# Autodesk Inventor assembly: Hand
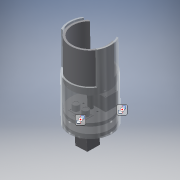
[picture p0: Inventor's stored thumbnail of the model, 180x180]
Saved by Autodesk Inventor 2016 (Build 200138000, 138)
## iProperties
Created: 2016-11-13
Part Number: Hand
Material: 一般
Document SubType Name: Assembly
Designer: Daisuke
Author: Daisuke
## Documents named in this file (10)
- C:\Users\Daisuke\Documents\GitHub\CAD\Hand\ver2\Hand.iam
- C:\Users\Daisuke\Documents\GitHub\CAD\Hand\ver2\Servo.iam
- C:\Users\Daisuke\Documents\GitHub\CAD\Hand\ver2\outsideBottom2.ipt
- C:\Users\Daisuke\Documents\GitHub\CAD\Hand\ver2\outsideBottom1.ipt
- C:\Users\Daisuke\Documents\GitHub\CAD\Hand\ver2\Servo.ipt
- C:\Users\Daisuke\Documents\GitHub\CAD\Hand\ver2\ServoArm.ipt
- C:\Users\Daisuke\Documents\GitHub\CAD\Hand\ver2\UFL08 -Housing.ipt
- C:\Users\Daisuke\Documents\GitHub\CAD\Hand\ver2\UltrasonicDistanceSencor.ipt
- C:\Users\Daisuke\Documents\GitHub\CAD\Hand\ver2\insideHand.iam
- C:\Users\Daisuke\Documents\GitHub\CAD\Hand\ver2\outsideCover1.ipt
## Components (9 placed, 8 different names)
1. Servo:1 [sub-assembly] — 挿入:1, 挿入:2, 挿入:3
2. outsideBottom2:1 — 挿入:9, 挿入:10, 挿入:11, メイト:1, メイト:4
3. outsideBottom1:1 — 挿入:1, 挿入:2, 挿入:3, 挿入:4, 挿入:5, 挿入:12, 挿入:13, メイト:2, メイト:3
4. Servo:2 — 挿入:8
5. ServoArm:1 — 挿入:8, 挿入:9, 挿入:10, 挿入:11
6. UFL08 -Housing:1 — 挿入:12, 挿入:13, 挿入:14
7. UltrasonicDistanceSencor:1 — 挿入:4, 挿入:5
8. insideHand:1 [sub-assembly] — 挿入:14
9. outsideCover1:1 — メイト:1, メイト:2, メイト:3, メイト:4
## Relationships (16: Insert 12, Mate 4)
- 挿入:1 [Insert]: Servo:1 ↔ outsideBottom1:1
- 挿入:2 [Insert]: Servo:1 ↔ outsideBottom1:1
- 挿入:3 [Insert]: Servo:1 ↔ outsideBottom1:1
- 挿入:4 [Insert]: outsideBottom1:1 ↔ UltrasonicDistanceSencor:1
- 挿入:5 [Insert]: outsideBottom1:1 ↔ UltrasonicDistanceSencor:1
- 挿入:8 [Insert] (0.5 mm): Servo:2 ↔ ServoArm:1
- 挿入:9 [Insert]: outsideBottom2:1 ↔ ServoArm:1
- 挿入:10 [Insert]: outsideBottom2:1 ↔ ServoArm:1
- 挿入:11 [Insert]: outsideBottom2:1 ↔ ServoArm:1
- 挿入:12 [Insert]: outsideBottom1:1 ↔ UFL08 -Housing:1
- 挿入:13 [Insert]: outsideBottom1:1 ↔ UFL08 -Housing:1
- 挿入:14 [Insert]: UFL08 -Housing:1 ↔ insideHand:1
- メイト:1 [Mate]: outsideBottom2:1 ↔ outsideCover1:1
- メイト:2 [Mate]: outsideBottom1:1 ↔ outsideCover1:1
- メイト:3 [Mate]: outsideBottom1:1 ↔ outsideCover1:1
- メイト:4 [Mate]: outsideBottom2:1 ↔ outsideCover1:1
